# Autodesk Inventor assembly: Assembly_WindTurbine
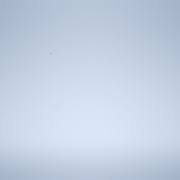
[picture p0: Inventor's stored thumbnail of the model, 180x180]
Saved by Autodesk Inventor 2021 (Build 250183000, 183)
## iProperties
Created: 2022-01-12
Part Number: Assembly_WindTurbine
Document SubType Name: Assembly
Designer: stefi
Author: stefi
## Documents named in this file (10)
- E:\Lavoro\Inventor\WindTurbine\Assembly_WindTurbine.iam
- E:\Lavoro\Inventor\WindTurbine\WindTurbine.ipt
- E:\Lavoro\Inventor\WindTurbine\Must.ipt
- E:\Lavoro\Inventor\WindTurbine\Housing.ipt
- E:\Lavoro\Inventor\WindTurbine\Rotor.ipt
- E:\Lavoro\Inventor\WindTurbine\Blades.ipt
- E:\Lavoro\Inventor\WindTurbine\Housing_MIR1.ipt
- E:\Lavoro\Inventor\WindTurbine\Washer.ipt
- E:\Lavoro\Inventor\WindTurbine\Shaft.ipt
- E:\Lavoro\Inventor\WindTurbine\Washer_MIR.ipt
## Components (12 placed, 9 different names)
1. WindTurbine:1 — Mate:2, Mate:14
2. Must:1 — Mate:1, Mate:4, Mate:14
3. Housing:1 — Mate:44, Mate:45, Mate:47, Mate:48
4. Rotor:1 — Mate:18, Mate:21, Mate:22, Rotation:1, Rotation:2, Rotation:3, Mate:38, Insert:1, Mate:41, Mate:42
5. Blades:2
6. Housing_MIR1:1 — Mate:31, Mate:32, Mate:33, Mate:34, Mate:35, Mate:36, Mate:37, Mate:47, Mate:48
7. Washer:1 — Mate:39, Mate:42, Flush:1
8. Shaft:1 — Mate:38, Insert:1, Flush:1, Insert:2
9. Washer_MIR:1 — Mate:43, Insert:2
10. Blades:1 — Mate:19, Mate:21, Rotation:2
11. Blades:3
12. Blades:4
## Component patterns: (3 elements, first: Blades:1)
## Relationships (34: Mate 28, RelateRotation 3, Insert 2, Flush 1)
- Mate:1: Must:1
- Mate:2: WindTurbine:1
- Mate:4: Must:1
- Mate:9
- Mate:14: WindTurbine:1 ↔ Must:1
- Mate:18: Rotor:1
- Mate:19: Blades:1
- Mate:20
- Mate:21: Rotor:1 ↔ Blades:1
- Mate:22: Rotor:1
- Mate:30
- Mate:31: Housing_MIR1:1
- Mate:32: Housing_MIR1:1
- Mate:33: Housing_MIR1:1
- Mate:34: Housing_MIR1:1
- Mate:35: Housing_MIR1:1
- Mate:36: Housing_MIR1:1
- Mate:37: Housing_MIR1:1
- Rotation:1 [RelateRotation] (1 ul): Rotor:1
- Rotation:2 [RelateRotation] (1 ul): Rotor:1 ↔ Blades:1
- Rotation:3 [RelateRotation] (1 ul): Rotor:1
- Mate:38: Rotor:1 ↔ Shaft:1
- Mate:39: Washer:1
- Insert:1: Rotor:1 ↔ Shaft:1
- Mate:41: Rotor:1
- Mate:42: Rotor:1 ↔ Washer:1
- Flush:1: Washer:1 ↔ Shaft:1
- Mate:43: Washer_MIR:1
- Insert:2: Shaft:1 ↔ Washer_MIR:1
- Mate:44: Housing:1
- Mate:45: Housing:1
- Mate:46
- Mate:47: Housing:1 ↔ Housing_MIR1:1
- Mate:48: Housing:1 ↔ Housing_MIR1:1
